# Autodesk Inventor assembly: E005-Bielle
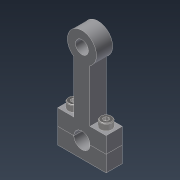
[picture p0: Inventor's stored thumbnail of the model, 180x180]
Saved by Autodesk Inventor 2021.3 (Build 253353000, 353)
## iProperties
Created: 2022-03-31
Part Number: E005-Bielle
Document SubType Name: Assembly
Designer: remi
Author: remi
## Documents named in this file (4)
- C:\Users\remi\OneDrive\Documents\Cours\05-HEVS\S2fb\mechanic\CCo\project\Compressor\E005-Bielle.iam
- C:\Users\remi\OneDrive\Documents\Cours\05-HEVS\S2fb\mechanic\CCo\project\Compressor\P012-Corps_bielle.ipt
- C:\Users\remi\OneDrive\Documents\Cours\05-HEVS\S2fb\mechanic\CCo\project\Compressor\P014-Chapeau_bielle.ipt
- C:\Users\remi\OneDrive\Documents\Inventor\Content Center Files\R2021\en-US\AS 1420\AS 1420 - 1973 - M4 x 20.ipt
## Components (4 placed, 3 different names)
1. P012-Corps_bielle:1 — Mate:1, Mate:2, Mate:3, Insert:1, Insert:2
2. P014-Chapeau_bielle:1 — Mate:1, Mate:2, Mate:3
3. AS 1420 - Metric M4 x 20:1 — Insert:1
4. AS 1420 - Metric M4 x 20:2 — Insert:2
## Relationships (5: Mate 3, Insert 2)
- Mate:1: P012-Corps_bielle:1 ↔ P014-Chapeau_bielle:1
- Mate:2: P012-Corps_bielle:1 ↔ P014-Chapeau_bielle:1
- Mate:3: P012-Corps_bielle:1 ↔ P014-Chapeau_bielle:1
- Insert:1: P012-Corps_bielle:1 ↔ AS 1420 - Metric M4 x 20:1
- Insert:2: P012-Corps_bielle:1 ↔ AS 1420 - Metric M4 x 20:2
